# Autodesk Inventor assembly: WristAssembly
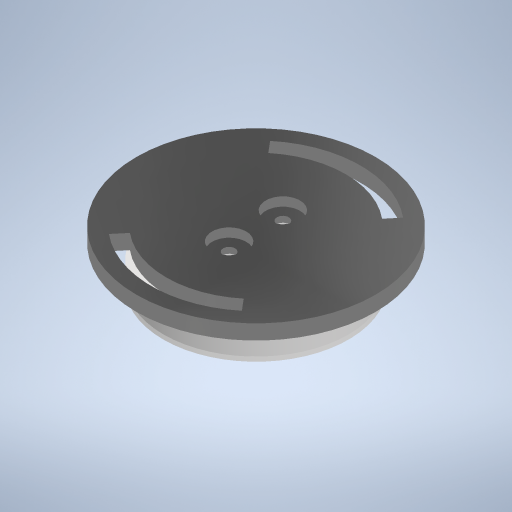
[picture p0: Inventor's stored thumbnail of the model, 512x512]
Saved by Autodesk Inventor 2023 (Build 270158000, 158)
## iProperties
Created: 2023-04-09
Part Number: WristAssembly
Document SubType Name: Assembly
Designer: adity
Author: adity
## Documents named in this file (4)
- C:\Users\adity\Downloads\Inventor\Robotic Wrist-Forearm\WristAssembly.iam
- C:\Users\adity\Downloads\Inventor\Robotic Wrist-Forearm\Wrist-Bearing Attachment.ipt
- C:\Users\adity\Downloads\Inventor\Robotic Wrist-Forearm\Wrist_Arm.ipt
- C:\Users\adity\Downloads\Inventor\Robotic Wrist-Forearm\Bearing.ipt
## Components (3 placed, 3 different names)
1. Wrist_Arm:1 — Insert:1
2. Wrist-Bearing Attachment:2 — Insert:1, Insert:2
3. Bearing:1 — Insert:2
## Relationships (2: Insert 2)
- Insert:1: Wrist_Arm:1 ↔ Wrist-Bearing Attachment:2
- Insert:2: Wrist-Bearing Attachment:2 ↔ Bearing:1
